# Autodesk Inventor assembly: Drive Base
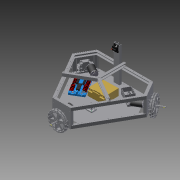
[picture p0: Inventor's stored thumbnail of the model, 180x180]
Saved by Autodesk Inventor 2013 (Build 170138000, 138)
## iProperties
Created: 2013-01-12
Part Number: Drive Base
Document SubType Name: Assembly
Designer: carneeki
Author: carneeki
## Documents named in this file (16)
- C:\Users\carneeki\Desktop\Kiwi Robot\Drive Base.iam
- C:\Users\carneeki\Desktop\Kiwi Robot\24in C-Channel.ipt
- C:\Users\carneeki\Desktop\Kiwi Robot\8in C-Channel.ipt
- C:\Users\carneeki\Desktop\Kiwi Robot\8in C-Channel - Vertical.ipt
- C:\Users\carneeki\Desktop\Kiwi Robot\C-Channel - Cross Support - Lower.ipt
- C:\Users\carneeki\Desktop\Kiwi Robot\Top Plate.ipt
- C:\Users\carneeki\Desktop\Kiwi Robot\Imported Components\ELEC\battery.ipt
- C:\Users\carneeki\Desktop\Kiwi Robot\Imported Components\ELEC\Breaker\Breaker.iam
- C:\Users\carneeki\Desktop\Kiwi Robot\Base Plate.ipt
- C:\Users\carneeki\Desktop\Kiwi Robot\HexShaft+Toughbox-mini.iam
- C:\Users\carneeki\Desktop\Kiwi Robot\Imported Components\ELEC\Battery Base.ipt
- C:\Users\carneeki\Desktop\Kiwi Robot\Imported Components\ELEC\cu_crio-9075_4-slot.ipt
- C:\Users\carneeki\Desktop\Kiwi Robot\Imported Components\PowerDistroBoard\PowerDistroBoard.iam
- C:\Users\carneeki\Desktop\Kiwi Robot\Imported Components\Victor884\Victor884.iam
- C:\Users\carneeki\Desktop\Kiwi Robot\15in c channel.ipt
- C:\Users\carneeki\Desktop\Kiwi Robot\C-Channel - Cross Support - Upper.ipt
## Components (37 placed, 30 different names)
1. Top Plate:1 — Mate:187, Mate:188, Mate:189, Mate:190
2. Base Plate:1 — Mate:167, Mate:168, Mate:169, Mate:170, Mate:180, Mate:181, Mate:182, Mate:185, Mate:192, Mate:203
3. 15in c channel:1 — Mate:199, Flush:146, Flush:147, Mate:201, Flush:148, Mate:203, Flush:149
4. 15in c channel:2 — Mate:199, Flush:146, Flush:147, Mate:200, Mate:202, Mate:204, Mate:205
5. 24in C-Channel:Back Edge:Lower — Mate:124, Flush:125, Mate:125, Mate:126, Mate:127, Flush:126, Mate:170
6. 8in C-Channel:Front Corner:Lower — Flush:128, Mate:130, Mate:131, Flush:129, Mate:132, Mate:133, Mate:134, Mate:135, Flush:130, Mate:177
7. 8in C-Channel:Left Corner:Lower — Mate:126, Mate:127, Flush:126, Mate:128, Mate:129, Flush:127, Mate:137, Flush:131, Mate:138, Mate:139, Flush:132, Mate:140, Flush:145
8. 24in C-Channel:Left Edge:Lower — Mate:128, Mate:129, Flush:127, Flush:128, Mate:130, Mate:136, Flush:140, Mate:169
9. 8in C-Channel:Right Corner:Lower — Mate:122, Mate:123, Flush:52, Mate:124, Mate:125, Mate:141, Flush:133, Mate:142, Mate:143, Flush:134, Mate:144
10. 24in C-Channel:Right Edge:Lower — Flush:50, Mate:120, Flush:51, Mate:121, Mate:122, Mate:123, Flush:52, Mate:131, Flush:129, Mate:168
11. 24in C-Channel:Back Edge:Upper — Mate:149, Flush:135, Mate:150, Mate:151, Mate:152, Flush:136, Mate:153, Mate:174, Mate:190, Mate:204, Insert:3, Flush:153
12. 8in C-Channel:Front Corner:Upper — Mate:159, Flush:138, Mate:160, Mate:161, Mate:162, Mate:163, Mate:164, Flush:139, Mate:176
13. 8in C-Channel:Left Corner:Upper — Mate:152, Flush:136, Mate:153, Mate:154, Mate:155, Mate:156, Flush:137, Mate:157, Mate:178, Flush:144, Mate:179
14. 24in C-Channel:Left Edge:Upper — Mate:156, Flush:137, Mate:157, Mate:158, Mate:159, Flush:138, Mate:160, Mate:187, Mate:188, Insert:1, Flush:151
15. 8in C-Channel:Right Corner:Upper — Mate:145, Mate:146, Mate:147, Mate:148, Mate:149, Flush:135, Mate:150, Mate:165, Mate:171, Mate:172, Mate:174
16. 24in C-Channel:Right Edge:Upper — Mate:163, Mate:164, Flush:139, Mate:165, Mate:166, Mate:173, Mate:189, Insert:2, Flush:150
17. 8in C-Channel - Vertical:Left 1 — Mate:139, Flush:132, Mate:140, Mate:151
18. 8in C-Channel - Vertical:Left 2 — Mate:137, Flush:131, Mate:138, Mate:154, Mate:155
19. 8in C-Channel - Vertical:Front 1 — Mate:135, Mate:136, Flush:130, Mate:158, Mate:175
20. 8in C-Channel - Vertical:Front 2 — Mate:132, Mate:133, Mate:134, Mate:161, Mate:162
21. 8in C-Channel - Vertical:Right 1 — Mate:141, Flush:133, Mate:142, Mate:146, Mate:147, Mate:166
22. 8in C-Channel - Vertical:Right 2 — Mate:143, Flush:134, Mate:144, Mate:145, Mate:148
23. HexShaft+Toughbox-mini:3 [sub-assembly] — Mate:175, Mate:176, Mate:177
24. HexShaft+Toughbox-mini:1 [sub-assembly] — Mate:178, Flush:144, Mate:179, Flush:145
25. HexShaft+Toughbox-mini:2 [sub-assembly] — Mate:171, Mate:172, Mate:173
26. Victor884:1 [sub-assembly]
27. battery:1 — Mate:184, Mate:185, Mate:186
28. Breaker:1 [sub-assembly] — Mate:200, Mate:201, Mate:202, Flush:148, Flush:149
29. PowerDistroBoard:1 [sub-assembly]
30. cu_crio-9075_4-slot:1 — Mate:192
31. Battery Base:1 — Mate:180, Mate:181, Mate:182, Mate:184, Mate:186
32. C-Channel - Cross Support - Upper:1 — Insert:1, Flush:151, Flush:152, Flush:154
33. C-Channel - Cross Support - Upper:2 — Insert:2, Flush:150, Flush:152
34. C-Channel - Cross Support - Upper:3 — Insert:3, Flush:153, Flush:154, Mate:205
35. C-Channel - Cross Support Lower:1 — Mate:116, Mate:117, Mate:119, Flush:50, Mate:120, Flush:51, Mate:121, Flush:142, Flush:143, Mate:167
36. C-Channel - Cross Support Lower:2 — Mate:116, Mate:117, Mate:118, Flush:125, Flush:141, Flush:143
37. C-Channel - Cross Support Lower:3 — Mate:118, Mate:119, Flush:140, Flush:141, Flush:142
## Relationships (120: Mate 84, Flush 33, Insert 3)
- Mate:116: C-Channel - Cross Support Lower:1 ↔ C-Channel - Cross Support Lower:2
- Mate:117: C-Channel - Cross Support Lower:1 ↔ C-Channel - Cross Support Lower:2
- Mate:118: C-Channel - Cross Support Lower:2 ↔ C-Channel - Cross Support Lower:3
- Mate:119: C-Channel - Cross Support Lower:1 ↔ C-Channel - Cross Support Lower:3
- Flush:50: 24in C-Channel:Right Edge:Lower ↔ C-Channel - Cross Support Lower:1
- Mate:120: 24in C-Channel:Right Edge:Lower ↔ C-Channel - Cross Support Lower:1
- Flush:51: 24in C-Channel:Right Edge:Lower ↔ C-Channel - Cross Support Lower:1
- Mate:121 (277.8633 mm): 24in C-Channel:Right Edge:Lower ↔ C-Channel - Cross Support Lower:1
- Mate:122: 8in C-Channel:Right Corner:Lower ↔ 24in C-Channel:Right Edge:Lower
- Mate:123: 8in C-Channel:Right Corner:Lower ↔ 24in C-Channel:Right Edge:Lower
- Flush:52: 8in C-Channel:Right Corner:Lower ↔ 24in C-Channel:Right Edge:Lower
- Mate:124: 24in C-Channel:Back Edge:Lower ↔ 8in C-Channel:Right Corner:Lower
- Flush:125: 24in C-Channel:Back Edge:Lower ↔ C-Channel - Cross Support Lower:2
- Mate:125: 24in C-Channel:Back Edge:Lower ↔ 8in C-Channel:Right Corner:Lower
- Mate:126: 24in C-Channel:Back Edge:Lower ↔ 8in C-Channel:Left Corner:Lower
- Mate:127: 24in C-Channel:Back Edge:Lower ↔ 8in C-Channel:Left Corner:Lower
- Flush:126: 24in C-Channel:Back Edge:Lower ↔ 8in C-Channel:Left Corner:Lower
- Mate:128: 8in C-Channel:Left Corner:Lower ↔ 24in C-Channel:Left Edge:Lower
- Mate:129: 8in C-Channel:Left Corner:Lower ↔ 24in C-Channel:Left Edge:Lower
- Flush:127: 8in C-Channel:Left Corner:Lower ↔ 24in C-Channel:Left Edge:Lower
- Flush:128: 8in C-Channel:Front Corner:Lower ↔ 24in C-Channel:Left Edge:Lower
- Mate:130: 8in C-Channel:Front Corner:Lower ↔ 24in C-Channel:Left Edge:Lower
- Mate:131: 8in C-Channel:Front Corner:Lower ↔ 24in C-Channel:Right Edge:Lower
- Flush:129: 8in C-Channel:Front Corner:Lower ↔ 24in C-Channel:Right Edge:Lower
- Mate:132: 8in C-Channel:Front Corner:Lower ↔ 8in C-Channel - Vertical:Front 2
- Mate:133: 8in C-Channel:Front Corner:Lower ↔ 8in C-Channel - Vertical:Front 2
- Mate:134: 8in C-Channel:Front Corner:Lower ↔ 8in C-Channel - Vertical:Front 2
- Mate:135: 8in C-Channel:Front Corner:Lower ↔ 8in C-Channel - Vertical:Front 1
- Mate:136: 24in C-Channel:Left Edge:Lower ↔ 8in C-Channel - Vertical:Front 1
- Flush:130: 8in C-Channel:Front Corner:Lower ↔ 8in C-Channel - Vertical:Front 1
- Mate:137: 8in C-Channel:Left Corner:Lower ↔ 8in C-Channel - Vertical:Left 2
- Flush:131: 8in C-Channel:Left Corner:Lower ↔ 8in C-Channel - Vertical:Left 2
- Mate:138: 8in C-Channel:Left Corner:Lower ↔ 8in C-Channel - Vertical:Left 2
- Mate:139: 8in C-Channel:Left Corner:Lower ↔ 8in C-Channel - Vertical:Left 1
- Flush:132: 8in C-Channel:Left Corner:Lower ↔ 8in C-Channel - Vertical:Left 1
- Mate:140: 8in C-Channel:Left Corner:Lower ↔ 8in C-Channel - Vertical:Left 1
- Mate:141: 8in C-Channel:Right Corner:Lower ↔ 8in C-Channel - Vertical:Right 1
- Flush:133: 8in C-Channel:Right Corner:Lower ↔ 8in C-Channel - Vertical:Right 1
- Mate:142: 8in C-Channel:Right Corner:Lower ↔ 8in C-Channel - Vertical:Right 1
- Mate:143: 8in C-Channel:Right Corner:Lower ↔ 8in C-Channel - Vertical:Right 2
- Flush:134: 8in C-Channel:Right Corner:Lower ↔ 8in C-Channel - Vertical:Right 2
- Mate:144: 8in C-Channel:Right Corner:Lower ↔ 8in C-Channel - Vertical:Right 2
- Mate:145: 8in C-Channel:Right Corner:Upper ↔ 8in C-Channel - Vertical:Right 2
- Mate:146: 8in C-Channel:Right Corner:Upper ↔ 8in C-Channel - Vertical:Right 1
- Mate:147: 8in C-Channel:Right Corner:Upper ↔ 8in C-Channel - Vertical:Right 1
- Mate:148: 8in C-Channel:Right Corner:Upper ↔ 8in C-Channel - Vertical:Right 2
- Mate:149: 24in C-Channel:Back Edge:Upper ↔ 8in C-Channel:Right Corner:Upper
- Flush:135: 24in C-Channel:Back Edge:Upper ↔ 8in C-Channel:Right Corner:Upper
- Mate:150: 24in C-Channel:Back Edge:Upper ↔ 8in C-Channel:Right Corner:Upper
- Mate:151: 24in C-Channel:Back Edge:Upper ↔ 8in C-Channel - Vertical:Left 1
- Mate:152: 24in C-Channel:Back Edge:Upper ↔ 8in C-Channel:Left Corner:Upper
- Flush:136: 24in C-Channel:Back Edge:Upper ↔ 8in C-Channel:Left Corner:Upper
- Mate:153: 24in C-Channel:Back Edge:Upper ↔ 8in C-Channel:Left Corner:Upper
- Mate:154: 8in C-Channel:Left Corner:Upper ↔ 8in C-Channel - Vertical:Left 2
- Mate:155: 8in C-Channel:Left Corner:Upper ↔ 8in C-Channel - Vertical:Left 2
- Mate:156: 8in C-Channel:Left Corner:Upper ↔ 24in C-Channel:Left Edge:Upper
- Flush:137: 8in C-Channel:Left Corner:Upper ↔ 24in C-Channel:Left Edge:Upper
- Mate:157: 8in C-Channel:Left Corner:Upper ↔ 24in C-Channel:Left Edge:Upper
- Mate:158: 24in C-Channel:Left Edge:Upper ↔ 8in C-Channel - Vertical:Front 1
- Mate:159: 8in C-Channel:Front Corner:Upper ↔ 24in C-Channel:Left Edge:Upper
- Flush:138: 8in C-Channel:Front Corner:Upper ↔ 24in C-Channel:Left Edge:Upper
- Mate:160: 8in C-Channel:Front Corner:Upper ↔ 24in C-Channel:Left Edge:Upper
- Mate:161: 8in C-Channel:Front Corner:Upper ↔ 8in C-Channel - Vertical:Front 2
- Mate:162: 8in C-Channel:Front Corner:Upper ↔ 8in C-Channel - Vertical:Front 2
- Mate:163: 8in C-Channel:Front Corner:Upper ↔ 24in C-Channel:Right Edge:Upper
- Mate:164: 8in C-Channel:Front Corner:Upper ↔ 24in C-Channel:Right Edge:Upper
- Flush:139: 8in C-Channel:Front Corner:Upper ↔ 24in C-Channel:Right Edge:Upper
- Mate:165: 8in C-Channel:Right Corner:Upper ↔ 24in C-Channel:Right Edge:Upper
- Mate:166: 24in C-Channel:Right Edge:Upper ↔ 8in C-Channel - Vertical:Right 1
- Flush:140: 24in C-Channel:Left Edge:Lower ↔ C-Channel - Cross Support Lower:3
- Flush:141: C-Channel - Cross Support Lower:2 ↔ C-Channel - Cross Support Lower:3
- Flush:142: C-Channel - Cross Support Lower:1 ↔ C-Channel - Cross Support Lower:3
- Flush:143: C-Channel - Cross Support Lower:1 ↔ C-Channel - Cross Support Lower:2
- Mate:167: Base Plate:1 ↔ C-Channel - Cross Support Lower:1
- Mate:168: Base Plate:1 ↔ 24in C-Channel:Right Edge:Lower
- Mate:169: Base Plate:1 ↔ 24in C-Channel:Left Edge:Lower
- Mate:170: Base Plate:1 ↔ 24in C-Channel:Back Edge:Lower
- Mate:171: 8in C-Channel:Right Corner:Upper ↔ HexShaft+Toughbox-mini:2
- Mate:172: 8in C-Channel:Right Corner:Upper ↔ HexShaft+Toughbox-mini:2
- Mate:173: 24in C-Channel:Right Edge:Upper ↔ HexShaft+Toughbox-mini:2
- Mate:174: 24in C-Channel:Back Edge:Upper ↔ 8in C-Channel:Right Corner:Upper
- Mate:175: 8in C-Channel - Vertical:Front 1 ↔ HexShaft+Toughbox-mini:3
- Mate:176: 8in C-Channel:Front Corner:Upper ↔ HexShaft+Toughbox-mini:3
- Mate:177: 8in C-Channel:Front Corner:Lower ↔ HexShaft+Toughbox-mini:3
- Mate:178: 8in C-Channel:Left Corner:Upper ↔ HexShaft+Toughbox-mini:1
- Flush:144: 8in C-Channel:Left Corner:Upper ↔ HexShaft+Toughbox-mini:1
- Mate:179: 8in C-Channel:Left Corner:Upper ↔ HexShaft+Toughbox-mini:1
- Flush:145: 8in C-Channel:Left Corner:Lower ↔ HexShaft+Toughbox-mini:1
- Mate:180: Base Plate:1 ↔ Battery Base:1
- Mate:181: Base Plate:1 ↔ Battery Base:1
- Mate:182: Base Plate:1 ↔ Battery Base:1
- Mate:184: battery:1 ↔ Battery Base:1
- Mate:185: Base Plate:1 ↔ battery:1
- Mate:186: battery:1 ↔ Battery Base:1
- Mate:187: Top Plate:1 ↔ 24in C-Channel:Left Edge:Upper
- Mate:188: Top Plate:1 ↔ 24in C-Channel:Left Edge:Upper
- Mate:189: Top Plate:1 ↔ 24in C-Channel:Right Edge:Upper
- Mate:190: Top Plate:1 ↔ 24in C-Channel:Back Edge:Upper
- [Mate]: Base Plate:1 ↔ PowerDistroBoard:1
- Mate:192: Base Plate:1 ↔ cu_crio-9075_4-slot:1
- [Mate]: Base Plate:1 ↔ Victor884:1
- Mate:199: 15in c channel:1 ↔ 15in c channel:2
- Flush:146: 15in c channel:1 ↔ 15in c channel:2
- Flush:147: 15in c channel:1 ↔ 15in c channel:2
- Mate:200: 15in c channel:2 ↔ Breaker:1
- Mate:201: 15in c channel:1 ↔ Breaker:1
- Mate:202: 15in c channel:2 ↔ Breaker:1
- Flush:148 (7.2644 mm): 15in c channel:1 ↔ Breaker:1
- Mate:203: Base Plate:1 ↔ 15in c channel:1
- Flush:149: 15in c channel:1 ↔ Breaker:1
- Mate:204: 15in c channel:2 ↔ 24in C-Channel:Back Edge:Upper
- Insert:1: 24in C-Channel:Left Edge:Upper ↔ C-Channel - Cross Support - Upper:1
- Insert:2: 24in C-Channel:Right Edge:Upper ↔ C-Channel - Cross Support - Upper:2
- Flush:150: 24in C-Channel:Right Edge:Upper ↔ C-Channel - Cross Support - Upper:2
- Flush:151: 24in C-Channel:Left Edge:Upper ↔ C-Channel - Cross Support - Upper:1
- Flush:152: C-Channel - Cross Support - Upper:1 ↔ C-Channel - Cross Support - Upper:2
- Insert:3: 24in C-Channel:Back Edge:Upper ↔ C-Channel - Cross Support - Upper:3
- Flush:153: 24in C-Channel:Back Edge:Upper ↔ C-Channel - Cross Support - Upper:3
- Flush:154: C-Channel - Cross Support - Upper:1 ↔ C-Channel - Cross Support - Upper:3
- Mate:205: 15in c channel:2 ↔ C-Channel - Cross Support - Upper:3
